# Autodesk Inventor assembly: Assembly_Trial_3
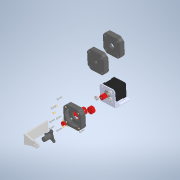
[picture p0: Inventor's stored thumbnail of the model, 180x180]
Saved by Autodesk Inventor 2022 (Build 260153000, 153)
## iProperties
Created: 2022-01-15
Part Number: Assembly_Trial_3
Document SubType Name: Assembly
Designer: Mlees
Author: Mlees
## Documents named in this file (14)
- C:\Users\Mlees\Desktop\504_Engineering\Stepper-Servo_Based_Robotic_Arm\Assembly_Trial_3.iam
- C:\Users\Mlees\Desktop\504_Engineering\Stepper-Servo_Based_Robotic_Arm\Downloaded Parts\nema17-speed-reducer-1.snapshot.9\24_Teeth_Sun_Gear.step.ipt
- C:\Users\Mlees\Desktop\504_Engineering\Stepper-Servo_Based_Robotic_Arm\Downloaded Parts\nema17-speed-reducer-1.snapshot.9\36_Teeth_Planet_Gear.step.ipt
- C:\Users\Mlees\Desktop\504_Engineering\Stepper-Servo_Based_Robotic_Arm\Downloaded Parts\nema17-speed-reducer-1.snapshot.9\96_Teeth_Gear.step.ipt
- C:\Users\Mlees\Desktop\504_Engineering\Stepper-Servo_Based_Robotic_Arm\Downloaded Parts\nema17-speed-reducer-1.snapshot.9\Gear_Cover.ipt
- C:\Users\Mlees\Desktop\504_Engineering\Stepper-Servo_Based_Robotic_Arm\Downloaded Parts\nema17-speed-reducer-1.snapshot.9\Plamet_Carrier.ipt
- C:\Users\Mlees\Desktop\504_Engineering\Stepper-Servo_Based_Robotic_Arm\Downloaded Parts\90751A113_18-8 Stainless Steel Socket Head Screws.ipt
- C:\Users\Mlees\Desktop\504_Engineering\Stepper-Servo_Based_Robotic_Arm\Downloaded Parts\nema-17-motor-mount-1.snapshot.1\NEMA_17_Bracket.ipt
- C:\Users\Mlees\Desktop\504_Engineering\Stepper-Servo_Based_Robotic_Arm\Downloaded Parts\nema17-speed-reducer-1.snapshot.9\Thread Insert M3 x 6mm v2.step.iam
- C:\Users\Mlees\Desktop\504_Engineering\Stepper-Servo_Based_Robotic_Arm\Downloaded Parts\Harmonic_Drive\Nema 17.ipt
- C:\Users\Mlees\Desktop\504_Engineering\Stepper-Servo_Based_Robotic_Arm\Downloaded Parts\nema17-speed-reducer-1.snapshot.9\Gear_Cover_modified.ipt
- C:\Users\Mlees\Desktop\504_Engineering\Stepper-Servo_Based_Robotic_Arm\Downloaded Parts\nema17-speed-reducer-1.snapshot.9\Plamet_Carrier_modified.ipt
- C:\Users\Mlees\Desktop\504_Engineering\Stepper-Servo_Based_Robotic_Arm\Created Parts\OutPut_Shaft_From_Gearbox.ipt
- C:\Users\Mlees\Desktop\504_Engineering\Stepper-Servo_Based_Robotic_Arm\Created Parts\604-2R2_Bearing4668K221_Permanently Lubricated Stainless Steel Ball Bearing.ipt
## Components (42 placed, 13 different names)
1. 24_Teeth_Sun_Gear.step:1 — Rotational:11
2. 36_Teeth_Planet_Gear.step:1
3. Gear_Cover:1
4. Plamet_Carrier:1
5. 90751A113_18-8 Stainless Steel Socket Head Screws:1
6. 90751A113_18-8 Stainless Steel Socket Head Screws:2
7. 90751A113_18-8 Stainless Steel Socket Head Screws:3
8. NEMA_17_Bracket:1 — Rigid:12
9. 36_Teeth_Planet_Gear.step:2
10. 36_Teeth_Planet_Gear.step:4
11. Thread Insert M3 x 6mm v2.step:1 [sub-assembly]
12. Thread Insert M3 x 6mm v2.step:2 [sub-assembly]
13. Thread Insert M3 x 6mm v2.step:3 [sub-assembly]
14. Thread Insert M3 x 6mm v2.step:4 [sub-assembly]
15. 90751A113_18-8 Stainless Steel Socket Head Screws:4
16. 90751A113_18-8 Stainless Steel Socket Head Screws:5
17. 90751A113_18-8 Stainless Steel Socket Head Screws:6
18. 90751A113_18-8 Stainless Steel Socket Head Screws:7
19. Nema 17:1 — Rigid:12, Rotational:11
20. 96_Teeth_Gear.step:2 — Rotational:12, Rotational:13, Rotational:14, Rotational:15, Rotational:16, Rotational:17, Rotational:18, Rotational:19
21. 90751A113_18-8 Stainless Steel Socket Head Screws:8 — Rotational:12
22. 90751A113_18-8 Stainless Steel Socket Head Screws:9 — Rotational:15
23. 90751A113_18-8 Stainless Steel Socket Head Screws:10 — Rotational:14
24. 90751A113_18-8 Stainless Steel Socket Head Screws:11 — Rotational:13
25. Thread Insert M3 x 6mm v2.step:5 [sub-assembly] — Rotational:16
26. Thread Insert M3 x 6mm v2.step:6 [sub-assembly] — Rotational:18
27. Thread Insert M3 x 6mm v2.step:7 [sub-assembly] — Rotational:19
28. Thread Insert M3 x 6mm v2.step:8 [sub-assembly] — Rotational:17
29. 24_Teeth_Sun_Gear.step:2
30. 36_Teeth_Planet_Gear.step:5
31. 36_Teeth_Planet_Gear.step:6
32. 36_Teeth_Planet_Gear.step:7
33. 90751A113_18-8 Stainless Steel Socket Head Screws:12
34. 90751A113_18-8 Stainless Steel Socket Head Screws:13
35. 90751A113_18-8 Stainless Steel Socket Head Screws:14
36. 90751A113_18-8 Stainless Steel Socket Head Screws:15
37. Gear_Cover_modified:1
38. Plamet_Carrier_modified:1
39. OutPut_Shaft_From_Gearbox:1
40. 604-2R2_Bearing4668K221_Permanently Lubricated Stainless Steel Ball Bearing:1
41. 604-2R2_Bearing4668K221_Permanently Lubricated Stainless Steel Ball Bearing:2
42. 604-2R2_Bearing4668K221_Permanently Lubricated Stainless Steel Ball Bearing:3
## Relationships (10: RevoluteJoint 9, WeldJoint 1)
- Rigid:12 [WeldJoint]: NEMA_17_Bracket:1 ↔ Nema 17:1
- Rotational:11 [RevoluteJoint]: 24_Teeth_Sun_Gear.step:1 ↔ Nema 17:1
- Rotational:12 [RevoluteJoint]: 96_Teeth_Gear.step:2 ↔ 90751A113_18-8 Stainless Steel Socket Head Screws:8
- Rotational:13 [RevoluteJoint]: 96_Teeth_Gear.step:2 ↔ 90751A113_18-8 Stainless Steel Socket Head Screws:11
- Rotational:14 [RevoluteJoint]: 96_Teeth_Gear.step:2 ↔ 90751A113_18-8 Stainless Steel Socket Head Screws:10
- Rotational:15 [RevoluteJoint]: 96_Teeth_Gear.step:2 ↔ 90751A113_18-8 Stainless Steel Socket Head Screws:9
- Rotational:16 [RevoluteJoint]: 96_Teeth_Gear.step:2 ↔ Thread Insert M3 x 6mm v2.step:5
- Rotational:17 [RevoluteJoint]: 96_Teeth_Gear.step:2 ↔ Thread Insert M3 x 6mm v2.step:8
- Rotational:18 [RevoluteJoint]: 96_Teeth_Gear.step:2 ↔ Thread Insert M3 x 6mm v2.step:6
- Rotational:19 [RevoluteJoint]: 96_Teeth_Gear.step:2 ↔ Thread Insert M3 x 6mm v2.step:7
